# Autodesk Inventor assembly: Baugruppe1
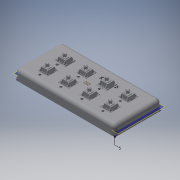
[picture p0: Inventor's stored thumbnail of the model, 180x180]
Saved by Autodesk Inventor 2019 (Build 230136000, 136)
## iProperties
Created: 2020-04-18
Part Number: Baugruppe1
Material: Generisch
Document SubType Name: Assembly
Designer: marc
Author: marc
## Documents named in this file (6)
- C:\Users\marc\Google Drive\Projekte\makroboard\makroboard_case\Baugruppe1.iam
- C:\Users\marc\Google Drive\Projekte\makroboard\makroboard_pcb\makroboard.iam
- C:\Users\marc\Google Drive\Projekte\makroboard\makroboard_pcb\1054500101.ipt
- C:\Users\marc\Google Drive\Projekte\makroboard\makroboard_pcb\asm_mx_asm_PCB.iam
- C:\Users\marc\Google Drive\Projekte\makroboard\makroboard_case\case_bot.ipt
- C:\Users\marc\Google Drive\Projekte\makroboard\makroboard_case\case_top.ipt
## Components (12 placed, 5 different names)
1. case_bot:1 — Fluchtend:1, Fluchtend:2, Fluchtend:3, Fluchtend:4, Fluchtend:5
2. case_top:1 — Fluchtend:4, Fluchtend:5
3. makroboard:1 [sub-assembly] — Starr:1, Starr:2, Starr:3, Starr:4, Starr:5, Starr:6, Starr:7, Drehbar:1, Starr:8, Fluchtend:1, Fluchtend:2, Fluchtend:3
4. 1054500101:1 — Starr:8
5. asm_mx_asm_PCB:1 [sub-assembly] — Starr:6
6. asm_mx_asm_PCB:2 [sub-assembly] — Starr:5
7. asm_mx_asm_PCB:3 [sub-assembly] — Starr:1
8. asm_mx_asm_PCB:4 [sub-assembly] — Starr:2
9. asm_mx_asm_PCB:5 [sub-assembly] — Starr:4
10. asm_mx_asm_PCB:6 [sub-assembly] — Drehbar:1
11. asm_mx_asm_PCB:7 [sub-assembly] — Starr:7
12. asm_mx_asm_PCB:8 [sub-assembly] — Starr:3
## Relationships (14: WeldJoint 8, Flush 5, RevoluteJoint 1)
- Starr:1 [WeldJoint] (-0.7 mm): makroboard:1 ↔ asm_mx_asm_PCB:3
- Starr:2 [WeldJoint]: makroboard:1 ↔ asm_mx_asm_PCB:4
- Starr:3 [WeldJoint]: makroboard:1 ↔ asm_mx_asm_PCB:8
- Starr:4 [WeldJoint]: makroboard:1 ↔ asm_mx_asm_PCB:5
- Starr:5 [WeldJoint]: makroboard:1 ↔ asm_mx_asm_PCB:2
- Starr:6 [WeldJoint]: makroboard:1 ↔ asm_mx_asm_PCB:1
- Starr:7 [WeldJoint]: makroboard:1 ↔ asm_mx_asm_PCB:7
- Drehbar:1 [RevoluteJoint] (-1.5 mm): makroboard:1 ↔ asm_mx_asm_PCB:6
- Starr:8 [WeldJoint]: makroboard:1 ↔ 1054500101:1
- Fluchtend:1 [Flush]: case_bot:1 ↔ makroboard:1
- Fluchtend:2 [Flush]: case_bot:1 ↔ makroboard:1
- Fluchtend:3 [Flush]: case_bot:1 ↔ makroboard:1
- Fluchtend:4 [Flush]: case_bot:1 ↔ case_top:1
- Fluchtend:5 [Flush]: case_bot:1 ↔ case_top:1
